# Autodesk Inventor assembly: joint_1_assembly
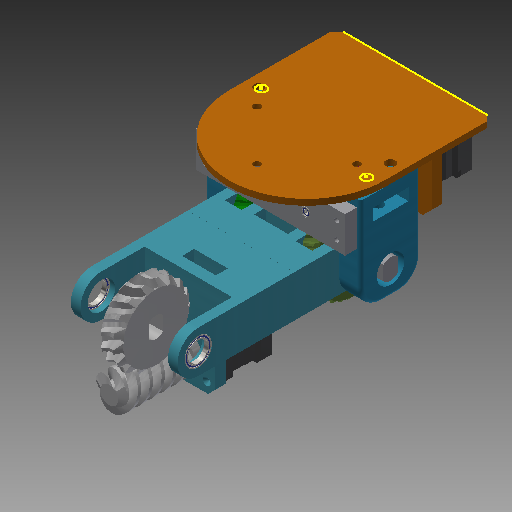
[picture p0: Inventor's stored thumbnail of the model, 512x512]
Saved by Autodesk Inventor 2019 (Build 230136000, 136)
## iProperties
Created: 2019-12-25
Part Number: joint_1_assembly
Material: Типовые
Document SubType Name: Assembly
Designer: Петров Иван
Author: Петров Иван
## Documents named in this file (13)
- E:\IVAN\Ivan_desktop\GitHub\Arm_manip\hardware\new\МД.001.300 - Звено 1.iam
- E:\IVAN\Ivan_desktop\GitHub\Arm_manip\hardware\new\МД.001.301 - Поворотный стол.ipt
- E:\IVAN\Ivan_desktop\GitHub\Arm_manip\hardware\Standart_things\Nema 17HS4401-S.ipt
- E:\IVAN\Ivan_desktop\GitHub\Arm_manip\hardware\Standart_things\Подшипник 17x23x4.ipt
- E:\IVAN\Ivan_desktop\GitHub\Arm_manip\hardware\new\МД.001.301- Стойка.ipt
- E:\IVAN\Ivan_desktop\GitHub\Arm_manip\hardware\new\МД.001.305 - Ось плеча.ipt
- E:\IVAN\Ivan_desktop\GitHub\Arm_manip\hardware\new\МД.001.400 - Червячная передача 1.iam
- E:\IVAN\Ivan_desktop\GitHub\Arm_manip\hardware\new\МД.001.500 - Червячная передача 2.iam
- E:\IVAN\Ivan_desktop\GitHub\Arm_manip\hardware\new\МД.001.302 - Фиксатор червей.ipt
- E:\IVAN\Ivan_desktop\GitHub\Arm_manip\hardware\Standart_things\Подшипник 4x8x3.ipt
- E:\IVAN\Ivan_desktop\GitHub\Arm_manip\hardware\new\МД.001.303 - 1-ая половина плеча.ipt
- E:\IVAN\Ivan_desktop\GitHub\Arm_manip\hardware\new\МД.001.304 - 2-ая половина плеча.ipt
- E:\IVAN\Ivan_desktop\GitHub\Arm_manip\hardware\new\МД.001.900 - Червяная передача 3.iam
## Components (22 placed, 10 different names)
1. МД.001.301 - Поворотный стол:1 — Совмещение:1, Совмещение:2, Совмещение:3, Совмещение:4, Совмещение:5, Совмещение:6, Заподлицо:1, Совмещение:7, Заподлицо:2, Совмещение:8, Совмещение:10, Совмещение:11, Заподлицо:3, Совмещение:12, Совмещение:13, Заподлицо:4, Угол:1, Угол:3
2. Nema 17HS4401-S:1 — Совмещение:1, Совмещение:2, Совмещение:3, Совмещение:33
3. Nema 17HS4401-S:2 — Совмещение:4, Совмещение:5, Совмещение:6, Совмещение:31
4. Подшипник 17x23x4:1 — Заподлицо:1, Совмещение:7
5. Подшипник 17x23x4:2 — Заподлицо:2, Совмещение:8
6. МД.001.301- Стойка:1 — Совмещение:10, Совмещение:11, Заподлицо:3, Заподлицо:5, Совмещение:14, Совмещение:36
7. МД.001.301- Стойка:2 — Совмещение:12, Совмещение:13, Заподлицо:4, Совмещение:16, Заподлицо:6, Совмещение:27, Заподлицо:7, Угол:2, Угол:8
8. Подшипник 17x23x4:3 — Совмещение:16, Заподлицо:6
9. Подшипник 17x23x4:4 — Заподлицо:5, Совмещение:14
10. МД.001.305 - Ось плеча:1 — Совмещение:27, Заподлицо:7, Совмещение:32, Совмещение:34, Совмещение:42, Совмещение:43, Совмещение:85, Совмещение:86
11. Червячная передача:1 [sub-assembly] — Совмещение:31, Угол:1, Совмещение:32, Угол:2, Совмещение:39, Совмещение:44, Совмещение:85
12. Червячная передача:2 [sub-assembly] — Совмещение:33, Угол:3, Совмещение:34, Совмещение:38, Совмещение:86
13. МД.001.302 - Фиксатор червей:1 — Совмещение:36, Совмещение:38, Совмещение:39, Совмещение:40, Заподлицо:8, Совмещение:41, Заподлицо:9
14. Подшипник 4x8x3:1 — Совмещение:40, Заподлицо:8
15. Подшипник 4x8x3:2 — Совмещение:41, Заподлицо:9
16. МД.001.303 - 1-ая половина плеча:1 — Совмещение:42, Совмещение:43, Совмещение:44, Совмещение:45, Совмещение:46, Совмещение:47, Угол:8
17. МД.001.304 - 2-ая половина плеча:1 — Совмещение:45, Совмещение:46, Совмещение:47, Совмещение:48, Угол:5, Угол:6, Совмещение:51, Заподлицо:11, Совмещение:52, Заподлицо:12, Совмещение:56, Совмещение:57, Совмещение:58, Совмещение:60
18. Nema 17HS4401-S:3 — Совмещение:48, Совмещение:50, Совмещение:56, Совмещение:57, Совмещение:58, Совмещение:59
19. Червячная передача:3 [sub-assembly] — Совмещение:50, Угол:5, Угол:6
20. Подшипник 17x23x4:5 — Совмещение:52, Заподлицо:12
21. Подшипник 17x23x4:6 — Совмещение:51, Заподлицо:11
22. Подшипник 17x23x4:7 — Совмещение:59, Совмещение:60
## Relationships (58: Mate 41, Flush 11, Angle 6)
- Совмещение:1 [Mate]: МД.001.301 - Поворотный стол:1 ↔ Nema 17HS4401-S:1
- Совмещение:2 [Mate]: МД.001.301 - Поворотный стол:1 ↔ Nema 17HS4401-S:1
- Совмещение:3 [Mate]: МД.001.301 - Поворотный стол:1 ↔ Nema 17HS4401-S:1
- Совмещение:4 [Mate]: МД.001.301 - Поворотный стол:1 ↔ Nema 17HS4401-S:2
- Совмещение:5 [Mate]: МД.001.301 - Поворотный стол:1 ↔ Nema 17HS4401-S:2
- Совмещение:6 [Mate]: МД.001.301 - Поворотный стол:1 ↔ Nema 17HS4401-S:2
- Заподлицо:1 [Flush]: МД.001.301 - Поворотный стол:1 ↔ Подшипник 17x23x4:1
- Совмещение:7 [Mate]: МД.001.301 - Поворотный стол:1 ↔ Подшипник 17x23x4:1
- Заподлицо:2 [Flush]: МД.001.301 - Поворотный стол:1 ↔ Подшипник 17x23x4:2
- Совмещение:8 [Mate]: МД.001.301 - Поворотный стол:1 ↔ Подшипник 17x23x4:2
- Совмещение:10 [Mate] (10 mm): МД.001.301 - Поворотный стол:1 ↔ МД.001.301- Стойка:1
- Совмещение:11 [Mate]: МД.001.301 - Поворотный стол:1 ↔ МД.001.301- Стойка:1
- Заподлицо:3 [Flush]: МД.001.301 - Поворотный стол:1 ↔ МД.001.301- Стойка:1
- Совмещение:12 [Mate]: МД.001.301 - Поворотный стол:1 ↔ МД.001.301- Стойка:2
- Совмещение:13 [Mate] (10 mm): МД.001.301 - Поворотный стол:1 ↔ МД.001.301- Стойка:2
- Заподлицо:4 [Flush]: МД.001.301 - Поворотный стол:1 ↔ МД.001.301- Стойка:2
- Заподлицо:5 [Flush]: МД.001.301- Стойка:1 ↔ Подшипник 17x23x4:4
- Совмещение:14 [Mate]: МД.001.301- Стойка:1 ↔ Подшипник 17x23x4:4
- Совмещение:16 [Mate]: МД.001.301- Стойка:2 ↔ Подшипник 17x23x4:3
- Заподлицо:6 [Flush]: МД.001.301- Стойка:2 ↔ Подшипник 17x23x4:3
- Совмещение:27 [Mate]: МД.001.301- Стойка:2 ↔ МД.001.305 - Ось плеча:1
- Заподлицо:7 [Flush]: МД.001.301- Стойка:2 ↔ МД.001.305 - Ось плеча:1
- Совмещение:31 [Mate]: Nema 17HS4401-S:2 ↔ Червячная передача:1
- Угол:1 [Angle] (0 deg): МД.001.301 - Поворотный стол:1 ↔ Червячная передача:1
- Совмещение:32 [Mate]: МД.001.305 - Ось плеча:1 ↔ Червячная передача:1
- Угол:2 [Angle] (0 deg): МД.001.301- Стойка:2 ↔ Червячная передача:1
- Совмещение:33 [Mate]: Nema 17HS4401-S:1 ↔ Червячная передача:2
- Угол:3 [Angle] (0 deg): МД.001.301 - Поворотный стол:1 ↔ Червячная передача:2
- Совмещение:34 [Mate]: МД.001.305 - Ось плеча:1 ↔ Червячная передача:2
- Совмещение:36 [Mate]: МД.001.301- Стойка:1 ↔ МД.001.302 - Фиксатор червей:1
- Совмещение:38 [Mate]: Червячная передача:2 ↔ МД.001.302 - Фиксатор червей:1
- Совмещение:39 [Mate]: Червячная передача:1 ↔ МД.001.302 - Фиксатор червей:1
- Совмещение:40 [Mate]: МД.001.302 - Фиксатор червей:1 ↔ Подшипник 4x8x3:1
- Заподлицо:8 [Flush]: МД.001.302 - Фиксатор червей:1 ↔ Подшипник 4x8x3:1
- Совмещение:41 [Mate]: МД.001.302 - Фиксатор червей:1 ↔ Подшипник 4x8x3:2
- Заподлицо:9 [Flush]: МД.001.302 - Фиксатор червей:1 ↔ Подшипник 4x8x3:2
- Совмещение:42 [Mate]: МД.001.305 - Ось плеча:1 ↔ МД.001.303 - 1-ая половина плеча:1
- Совмещение:43 [Mate]: МД.001.305 - Ось плеча:1 ↔ МД.001.303 - 1-ая половина плеча:1
- Совмещение:44 [Mate]: Червячная передача:1 ↔ МД.001.303 - 1-ая половина плеча:1
- Совмещение:45 [Mate]: МД.001.303 - 1-ая половина плеча:1 ↔ МД.001.304 - 2-ая половина плеча:1
- Совмещение:46 [Mate]: МД.001.303 - 1-ая половина плеча:1 ↔ МД.001.304 - 2-ая половина плеча:1
- Совмещение:47 [Mate]: МД.001.303 - 1-ая половина плеча:1 ↔ МД.001.304 - 2-ая половина плеча:1
- Совмещение:48 [Mate]: МД.001.304 - 2-ая половина плеча:1 ↔ Nema 17HS4401-S:3
- Совмещение:50 [Mate]: Nema 17HS4401-S:3 ↔ Червячная передача:3
- Угол:5 [Angle] (0 deg): МД.001.304 - 2-ая половина плеча:1 ↔ Червячная передача:3
- Угол:6 [Angle] (0 deg): МД.001.304 - 2-ая половина плеча:1 ↔ Червячная передача:3
- Совмещение:51 [Mate]: МД.001.304 - 2-ая половина плеча:1 ↔ Подшипник 17x23x4:6
- Заподлицо:11 [Flush]: МД.001.304 - 2-ая половина плеча:1 ↔ Подшипник 17x23x4:6
- Совмещение:52 [Mate]: МД.001.304 - 2-ая половина плеча:1 ↔ Подшипник 17x23x4:5
- Заподлицо:12 [Flush]: МД.001.304 - 2-ая половина плеча:1 ↔ Подшипник 17x23x4:5
- Совмещение:56 [Mate]: МД.001.304 - 2-ая половина плеча:1 ↔ Nema 17HS4401-S:3
- Совмещение:57 [Mate]: МД.001.304 - 2-ая половина плеча:1 ↔ Nema 17HS4401-S:3
- Совмещение:58 [Mate]: МД.001.304 - 2-ая половина плеча:1 ↔ Nema 17HS4401-S:3
- Совмещение:59 [Mate]: Nema 17HS4401-S:3 ↔ Подшипник 17x23x4:7
- Совмещение:60 [Mate]: МД.001.304 - 2-ая половина плеча:1 ↔ Подшипник 17x23x4:7
- Совмещение:85 [Mate]: МД.001.305 - Ось плеча:1 ↔ Червячная передача:1
- Совмещение:86 [Mate]: МД.001.305 - Ось плеча:1 ↔ Червячная передача:2
- Угол:8 [Angle] (0 deg): МД.001.301- Стойка:2 ↔ МД.001.303 - 1-ая половина плеча:1
